# Autodesk Inventor assembly: PowerS_cap
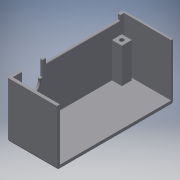
[picture p0: Inventor's stored thumbnail of the model, 180x180]
Saved by Autodesk Inventor 2019.3 (Build 233278000, 278)
## iProperties
Created: 2020-09-01
Part Number: PowerS_cap
Material: Generisch
Document SubType Name: Assembly
Designer: Nicolas Frick
Author: Nicolas Frick
## Documents named in this file (2)
- C:\Users\Nicolas Frick\Sync\OneDrive\airhockeybot\mechanical_design\common_cad_parts\print_models\PowerS_cap.iam
- C:\Users\Nicolas Frick\Sync\OneDrive\airhockeybot\mechanical_design\inventor\PowerS_cap.ipt
## Components (1 placed, 1 different names)
1. PowerS_cap:1 — Passend:1, Passend:2, Fluchtend:1
## Relationships (3: Mate 2, Flush 1)
- Passend:1 [Mate]: PowerS_cap:1
- Passend:2 [Mate]: PowerS_cap:1
- Fluchtend:1 [Flush]: PowerS_cap:1
